# Autodesk Inventor assembly: Full_Assembly
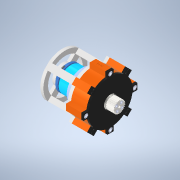
[picture p0: Inventor's stored thumbnail of the model, 180x180]
Saved by Autodesk Inventor 2022 (Build 260153000, 153)
## iProperties
Created: 2022-04-22
Part Number: Full_Assembly
Document SubType Name: Assembly
Designer: Mlees
Mass: 185.858 g
Surface Area: 506.5 cm^2
Volume: 64.9756 cm^3
Density: 2.86043 g/cm^3
Author: Mlees
## Documents named in this file (15)
- C:\Users\Mlees\Desktop\504Engineering\Project_0000\Designs\Design_2\Created_Parts\Full_Assembly.iam
- C:\Users\Mlees\Desktop\504Engineering\Project_0000\Designs\Design_2\Created_Parts\Gear_Box_Chasis_Lvl_1.ipt
- C:\Users\Mlees\Desktop\504Engineering\Project_0000\Designs\Design_2\Created_Parts\Gear_Box_Chasis_Divider.ipt
- C:\Users\Mlees\Desktop\504Engineering\Project_0000\Designs\Design_2\Created_Parts\Gear_Box_Motor_Input.ipt
- C:\Users\Mlees\Desktop\504Engineering\Project_0000\Designs\Design_2\Downloads\m100-motor-1.snapshot.1\M100-MOTOR-R1.ipt
- C:\Users\Mlees\Desktop\504Engineering\Project_0000\Designs\Design_2\Created_Parts\Gear_Folder\5to1GearCreation_Trial_1\Design Accelerator\Spur Gear23.ipt
- C:\Users\Mlees\Desktop\504Engineering\Project_0000\Designs\Design_2\Created_Parts\Planet_Gear_Output.ipt
- C:\Users\Mlees\Desktop\504Engineering\Project_0000\Designs\Design_2\Created_Parts\Gear_Box_Motor_Support_Bracket.ipt
- C:\Users\Mlees\Desktop\504Engineering\Project_0000\Designs\Design_2\Downloads\91420A014_Steel Phillips Flat Head Screws_M2-5x5mm.ipt
- C:\Users\Mlees\Desktop\504Engineering\Project_0000\Designs\Design_2\Downloads\91420A116_Steel Phillips Flat Head Screws_M3x6mm.ipt
- C:\Users\Mlees\Desktop\504Engineering\Project_0000\Designs\Design_2\Downloads\94180A321_Tapered Heat-Set Inserts for Plastic_M2-5x3.4mm_0-152inmaxhomesize.ipt
- C:\Users\Mlees\Desktop\504Engineering\Project_0000\Designs\Design_2\Downloads\91420A120_Steel Phillips Flat Head ScrewsM3x10mm.ipt
- C:\Users\Mlees\Desktop\504Engineering\Project_0000\Designs\Design_2\Created_Parts\Gear_Box_Second_Stage_Input.ipt
- C:\Users\Mlees\Desktop\504Engineering\Project_0000\Designs\Design_2\Downloads\94180A312_Tapered Heat-Set Inserts for Plastic_M2_2.7mmmaxholesize.ipt
- C:\Users\Mlees\Desktop\504Engineering\Project_0000\Designs\Design_2\Downloads\91420A006_Steel Phillips Flat Head ScrewsM2x12mm.ipt
## Components (43 placed, 12 different names)
1. Spur Gear2:1 — Mate:24, Mate:25, Flush:1, Flush:2, Flush:3, Mate:40, Mate:43, Mate:74, Mate:75, Mate:76, Mate:77, Mate:78, Mate:79, Mate:80, Mate:81, Mate:82, Mate:83, Mate:84, Mate:85, Mate:86, Mate:87, Mate:88, Mate:89, Mate:90, Mate:91, Mate:92, Mate:93
2. Gear_Box_Chasis_Divider:1 — Mate:43, Mate:92, Mate:93, Mate:122, Mate:123, Mate:124, Mate:125, Mate:126, Mate:127, Mate:128, Mate:129
3. Spur Gear1:1 — Mate:20, Mate:23, Mate:21, Mate:24, Mate:25, Mate:26, Mate:27, Mate:28, Mate:35, Rotation:1, Mate:62, Mate:63, Mate:64, Mate:65
4. M100-MOTOR-R1:1 — Mate:20, Mate:23, Mate:21
5. Spur Gear2:2 — Flush:3, Mate:27, Mate:36, Mate:98, Mate:99
6. Spur Gear2:3 — Flush:2, Mate:28, Mate:38, Mate:94, Mate:95
7. Spur Gear2:4 — Flush:1, Mate:26, Mate:37, Mate:39, Mate:96, Mate:97
8. Planet_Gear_Output:1 — Mate:35, Mate:36, Mate:37, Mate:38, Mate:39, Rotation:1, Mate:103, Mate:104, Mate:105, Mate:106, Mate:107, Mate:108, Mate:109, Mate:110
9. Gear_Box_Motor_Support_Bracket:1 — Mate:40, Mate:55, Mate:57, Mate:59, Mate:61, Mate:66, Mate:67, Mate:68, Mate:69, Mate:70, Mate:71, Mate:72, Mate:73, Mate:90, Mate:91
10. 91420A014_Steel Phillips Flat Head Screws_M2-5x5mm:5 — Mate:55
11. 91420A014_Steel Phillips Flat Head Screws_M2-5x5mm:6 — Mate:59
12. 91420A014_Steel Phillips Flat Head Screws_M2-5x5mm:7 — Mate:61
13. 91420A014_Steel Phillips Flat Head Screws_M2-5x5mm:8 — Mate:57
14. 91420A116_Steel Phillips Flat Head Screws_M3x6mm:1 — Mate:67, Mate:71
15. 91420A116_Steel Phillips Flat Head Screws_M3x6mm:2 — Mate:62, Mate:63
16. 91420A116_Steel Phillips Flat Head Screws_M3x6mm:3 — Mate:64, Mate:65
17. 91420A116_Steel Phillips Flat Head Screws_M3x6mm:4 — Mate:66, Mate:72
18. 91420A116_Steel Phillips Flat Head Screws_M3x6mm:5 — Mate:69, Mate:73
19. 91420A116_Steel Phillips Flat Head Screws_M3x6mm:6 — Mate:68, Mate:70
20. 94180A321_Tapered Heat-Set Inserts for Plastic_M2-5x3.4mm_0-152inmaxhomesize:1 — Mate:74, Mate:75
21. 94180A321_Tapered Heat-Set Inserts for Plastic_M2-5x3.4mm_0-152inmaxhomesize:2 — Mate:83, Mate:88
22. 94180A321_Tapered Heat-Set Inserts for Plastic_M2-5x3.4mm_0-152inmaxhomesize:3 — Mate:82, Mate:87
23. 94180A321_Tapered Heat-Set Inserts for Plastic_M2-5x3.4mm_0-152inmaxhomesize:4 — Mate:78, Mate:79
24. 94180A321_Tapered Heat-Set Inserts for Plastic_M2-5x3.4mm_0-152inmaxhomesize:5 — Mate:80, Mate:81
25. 94180A321_Tapered Heat-Set Inserts for Plastic_M2-5x3.4mm_0-152inmaxhomesize:6 — Mate:84, Mate:89
26. 94180A321_Tapered Heat-Set Inserts for Plastic_M2-5x3.4mm_0-152inmaxhomesize:7 — Mate:85, Mate:86
27. 94180A321_Tapered Heat-Set Inserts for Plastic_M2-5x3.4mm_0-152inmaxhomesize:8 — Mate:76, Mate:77
28. 91420A120_Steel Phillips Flat Head ScrewsM3x10mm:1 — Mate:98, Mate:99
29. 91420A120_Steel Phillips Flat Head ScrewsM3x10mm:2 — Mate:94, Mate:95
30. 91420A120_Steel Phillips Flat Head ScrewsM3x10mm:3 — Mate:96, Mate:97
31. Spur Gear1:2 — Mate:111, Mate:112, Mate:113, Mate:114, Mate:115, Mate:116, Mate:117, Mate:118, Mate:119, Mate:120, Mate:121
32. 94180A312_Tapered Heat-Set Inserts for Plastic_M2_2.7mmmaxholesize:1 — Mate:103, Mate:108, Mate:111
33. 94180A312_Tapered Heat-Set Inserts for Plastic_M2_2.7mmmaxholesize:2 — Mate:106, Mate:110, Mate:112, Mate:113
34. 94180A312_Tapered Heat-Set Inserts for Plastic_M2_2.7mmmaxholesize:3 — Mate:104, Mate:107
35. 94180A312_Tapered Heat-Set Inserts for Plastic_M2_2.7mmmaxholesize:4 — Mate:105, Mate:109
36. 91420A006_Steel Phillips Flat Head ScrewsM2x12mm:1 — Mate:114, Mate:121
37. 91420A006_Steel Phillips Flat Head ScrewsM2x12mm:2 — Mate:115, Mate:120
38. 91420A006_Steel Phillips Flat Head ScrewsM2x12mm:3 — Mate:116, Mate:118
39. 91420A006_Steel Phillips Flat Head ScrewsM2x12mm:4 — Mate:117, Mate:119
40. 91420A116_Steel Phillips Flat Head Screws_M3x6mm:7 — Mate:122, Mate:123
41. 91420A116_Steel Phillips Flat Head Screws_M3x6mm:8 — Mate:124, Mate:129
42. 91420A116_Steel Phillips Flat Head Screws_M3x6mm:9 — Mate:125, Mate:128
43. 91420A116_Steel Phillips Flat Head Screws_M3x6mm:10 — Mate:126, Mate:127
## Relationships (88: Mate 84, Flush 3, RelateRotation 1)
- Mate:20: Spur Gear1:1 ↔ M100-MOTOR-R1:1
- Mate:23: Spur Gear1:1 ↔ M100-MOTOR-R1:1
- Mate:21: Spur Gear1:1 ↔ M100-MOTOR-R1:1
- Mate:24: Spur Gear2:1 ↔ Spur Gear1:1
- Mate:25: Spur Gear2:1 ↔ Spur Gear1:1
- Flush:1: Spur Gear2:1 ↔ Spur Gear2:4
- Flush:2: Spur Gear2:1 ↔ Spur Gear2:3
- Flush:3: Spur Gear2:1 ↔ Spur Gear2:2
- Mate:26 (16.272 mm): Spur Gear1:1 ↔ Spur Gear2:4
- Mate:27 (16.272 mm): Spur Gear1:1 ↔ Spur Gear2:2
- Mate:28 (16.272 mm): Spur Gear1:1 ↔ Spur Gear2:3
- Mate:35: Spur Gear1:1 ↔ Planet_Gear_Output:1
- Mate:36: Spur Gear2:2 ↔ Planet_Gear_Output:1
- Mate:37: Spur Gear2:4 ↔ Planet_Gear_Output:1
- Mate:38: Spur Gear2:3 ↔ Planet_Gear_Output:1
- Mate:39: Spur Gear2:4 ↔ Planet_Gear_Output:1
- Rotation:1 [RelateRotation] (0.2 ul): Spur Gear1:1 ↔ Planet_Gear_Output:1
- Mate:40: Spur Gear2:1 ↔ Gear_Box_Motor_Support_Bracket:1
- Mate:43: Spur Gear2:1 ↔ Gear_Box_Chasis_Divider:1
- Mate:55: Gear_Box_Motor_Support_Bracket:1 ↔ 91420A014_Steel Phillips Flat Head Screws_M2-5x5mm:5
- Mate:57: Gear_Box_Motor_Support_Bracket:1 ↔ 91420A014_Steel Phillips Flat Head Screws_M2-5x5mm:8
- Mate:59: Gear_Box_Motor_Support_Bracket:1 ↔ 91420A014_Steel Phillips Flat Head Screws_M2-5x5mm:6
- Mate:61: Gear_Box_Motor_Support_Bracket:1 ↔ 91420A014_Steel Phillips Flat Head Screws_M2-5x5mm:7
- Mate:62: Spur Gear1:1 ↔ 91420A116_Steel Phillips Flat Head Screws_M3x6mm:2
- Mate:63: Spur Gear1:1 ↔ 91420A116_Steel Phillips Flat Head Screws_M3x6mm:2
- Mate:64: Spur Gear1:1 ↔ 91420A116_Steel Phillips Flat Head Screws_M3x6mm:3
- Mate:65: Spur Gear1:1 ↔ 91420A116_Steel Phillips Flat Head Screws_M3x6mm:3
- Mate:66: Gear_Box_Motor_Support_Bracket:1 ↔ 91420A116_Steel Phillips Flat Head Screws_M3x6mm:4
- Mate:67: Gear_Box_Motor_Support_Bracket:1 ↔ 91420A116_Steel Phillips Flat Head Screws_M3x6mm:1
- Mate:68: Gear_Box_Motor_Support_Bracket:1 ↔ 91420A116_Steel Phillips Flat Head Screws_M3x6mm:6
- Mate:69: Gear_Box_Motor_Support_Bracket:1 ↔ 91420A116_Steel Phillips Flat Head Screws_M3x6mm:5
- Mate:70: Gear_Box_Motor_Support_Bracket:1 ↔ 91420A116_Steel Phillips Flat Head Screws_M3x6mm:6
- Mate:71: Gear_Box_Motor_Support_Bracket:1 ↔ 91420A116_Steel Phillips Flat Head Screws_M3x6mm:1
- Mate:72: Gear_Box_Motor_Support_Bracket:1 ↔ 91420A116_Steel Phillips Flat Head Screws_M3x6mm:4
- Mate:73: Gear_Box_Motor_Support_Bracket:1 ↔ 91420A116_Steel Phillips Flat Head Screws_M3x6mm:5
- Mate:74: Spur Gear2:1 ↔ 94180A321_Tapered Heat-Set Inserts for Plastic_M2-5x3.4mm_0-152inmaxhomesize:1
- Mate:75: Spur Gear2:1 ↔ 94180A321_Tapered Heat-Set Inserts for Plastic_M2-5x3.4mm_0-152inmaxhomesize:1
- Mate:76: Spur Gear2:1 ↔ 94180A321_Tapered Heat-Set Inserts for Plastic_M2-5x3.4mm_0-152inmaxhomesize:8
- Mate:77: Spur Gear2:1 ↔ 94180A321_Tapered Heat-Set Inserts for Plastic_M2-5x3.4mm_0-152inmaxhomesize:8
- Mate:78: Spur Gear2:1 ↔ 94180A321_Tapered Heat-Set Inserts for Plastic_M2-5x3.4mm_0-152inmaxhomesize:4
- Mate:79: Spur Gear2:1 ↔ 94180A321_Tapered Heat-Set Inserts for Plastic_M2-5x3.4mm_0-152inmaxhomesize:4
- Mate:80: Spur Gear2:1 ↔ 94180A321_Tapered Heat-Set Inserts for Plastic_M2-5x3.4mm_0-152inmaxhomesize:5
- Mate:81: Spur Gear2:1 ↔ 94180A321_Tapered Heat-Set Inserts for Plastic_M2-5x3.4mm_0-152inmaxhomesize:5
- Mate:82: Spur Gear2:1 ↔ 94180A321_Tapered Heat-Set Inserts for Plastic_M2-5x3.4mm_0-152inmaxhomesize:3
- Mate:83: Spur Gear2:1 ↔ 94180A321_Tapered Heat-Set Inserts for Plastic_M2-5x3.4mm_0-152inmaxhomesize:2
- Mate:84: Spur Gear2:1 ↔ 94180A321_Tapered Heat-Set Inserts for Plastic_M2-5x3.4mm_0-152inmaxhomesize:6
- Mate:85: Spur Gear2:1 ↔ 94180A321_Tapered Heat-Set Inserts for Plastic_M2-5x3.4mm_0-152inmaxhomesize:7
- Mate:86: Spur Gear2:1 ↔ 94180A321_Tapered Heat-Set Inserts for Plastic_M2-5x3.4mm_0-152inmaxhomesize:7
- Mate:87: Spur Gear2:1 ↔ 94180A321_Tapered Heat-Set Inserts for Plastic_M2-5x3.4mm_0-152inmaxhomesize:3
- Mate:88: Spur Gear2:1 ↔ 94180A321_Tapered Heat-Set Inserts for Plastic_M2-5x3.4mm_0-152inmaxhomesize:2
- Mate:89: Spur Gear2:1 ↔ 94180A321_Tapered Heat-Set Inserts for Plastic_M2-5x3.4mm_0-152inmaxhomesize:6
- Mate:90: Spur Gear2:1 ↔ Gear_Box_Motor_Support_Bracket:1
- Mate:91: Spur Gear2:1 ↔ Gear_Box_Motor_Support_Bracket:1
- Mate:92: Spur Gear2:1 ↔ Gear_Box_Chasis_Divider:1
- Mate:93: Spur Gear2:1 ↔ Gear_Box_Chasis_Divider:1
- Mate:94: Spur Gear2:3 ↔ 91420A120_Steel Phillips Flat Head ScrewsM3x10mm:2
- Mate:95: Spur Gear2:3 ↔ 91420A120_Steel Phillips Flat Head ScrewsM3x10mm:2
- Mate:96: Spur Gear2:4 ↔ 91420A120_Steel Phillips Flat Head ScrewsM3x10mm:3
- Mate:97: Spur Gear2:4 ↔ 91420A120_Steel Phillips Flat Head ScrewsM3x10mm:3
- Mate:98: Spur Gear2:2 ↔ 91420A120_Steel Phillips Flat Head ScrewsM3x10mm:1
- Mate:99: Spur Gear2:2 ↔ 91420A120_Steel Phillips Flat Head ScrewsM3x10mm:1
- Mate:103: Planet_Gear_Output:1 ↔ 94180A312_Tapered Heat-Set Inserts for Plastic_M2_2.7mmmaxholesize:1
- Mate:104: Planet_Gear_Output:1 ↔ 94180A312_Tapered Heat-Set Inserts for Plastic_M2_2.7mmmaxholesize:3
- Mate:105: Planet_Gear_Output:1 ↔ 94180A312_Tapered Heat-Set Inserts for Plastic_M2_2.7mmmaxholesize:4
- Mate:106: Planet_Gear_Output:1 ↔ 94180A312_Tapered Heat-Set Inserts for Plastic_M2_2.7mmmaxholesize:2
- Mate:107: Planet_Gear_Output:1 ↔ 94180A312_Tapered Heat-Set Inserts for Plastic_M2_2.7mmmaxholesize:3
- Mate:108: Planet_Gear_Output:1 ↔ 94180A312_Tapered Heat-Set Inserts for Plastic_M2_2.7mmmaxholesize:1
- Mate:109: Planet_Gear_Output:1 ↔ 94180A312_Tapered Heat-Set Inserts for Plastic_M2_2.7mmmaxholesize:4
- Mate:110: Planet_Gear_Output:1 ↔ 94180A312_Tapered Heat-Set Inserts for Plastic_M2_2.7mmmaxholesize:2
- Mate:111: Spur Gear1:2 ↔ 94180A312_Tapered Heat-Set Inserts for Plastic_M2_2.7mmmaxholesize:1
- Mate:112: Spur Gear1:2 ↔ 94180A312_Tapered Heat-Set Inserts for Plastic_M2_2.7mmmaxholesize:2
- Mate:113: Spur Gear1:2 ↔ 94180A312_Tapered Heat-Set Inserts for Plastic_M2_2.7mmmaxholesize:2
- Mate:114: Spur Gear1:2 ↔ 91420A006_Steel Phillips Flat Head ScrewsM2x12mm:1
- Mate:115: Spur Gear1:2 ↔ 91420A006_Steel Phillips Flat Head ScrewsM2x12mm:2
- Mate:116: Spur Gear1:2 ↔ 91420A006_Steel Phillips Flat Head ScrewsM2x12mm:3
- Mate:117: Spur Gear1:2 ↔ 91420A006_Steel Phillips Flat Head ScrewsM2x12mm:4
- Mate:118: Spur Gear1:2 ↔ 91420A006_Steel Phillips Flat Head ScrewsM2x12mm:3
- Mate:119: Spur Gear1:2 ↔ 91420A006_Steel Phillips Flat Head ScrewsM2x12mm:4
- Mate:120: Spur Gear1:2 ↔ 91420A006_Steel Phillips Flat Head ScrewsM2x12mm:2
- Mate:121: Spur Gear1:2 ↔ 91420A006_Steel Phillips Flat Head ScrewsM2x12mm:1
- Mate:122: Gear_Box_Chasis_Divider:1 ↔ 91420A116_Steel Phillips Flat Head Screws_M3x6mm:7
- Mate:123: Gear_Box_Chasis_Divider:1 ↔ 91420A116_Steel Phillips Flat Head Screws_M3x6mm:7
- Mate:124: Gear_Box_Chasis_Divider:1 ↔ 91420A116_Steel Phillips Flat Head Screws_M3x6mm:8
- Mate:125: Gear_Box_Chasis_Divider:1 ↔ 91420A116_Steel Phillips Flat Head Screws_M3x6mm:9
- Mate:126: Gear_Box_Chasis_Divider:1 ↔ 91420A116_Steel Phillips Flat Head Screws_M3x6mm:10
- Mate:127: Gear_Box_Chasis_Divider:1 ↔ 91420A116_Steel Phillips Flat Head Screws_M3x6mm:10
- Mate:128: Gear_Box_Chasis_Divider:1 ↔ 91420A116_Steel Phillips Flat Head Screws_M3x6mm:9
- Mate:129: Gear_Box_Chasis_Divider:1 ↔ 91420A116_Steel Phillips Flat Head Screws_M3x6mm:8
